# Autodesk Inventor assembly: 000.003 - Блок АКБ СБ
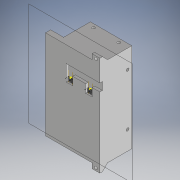
[picture p0: Inventor's stored thumbnail of the model, 180x180]
Saved by Autodesk Inventor 2022 (Build 260153000, 153)
## iProperties
Created: 2022-02-26
Part Number: 000.003 - Блок АКБ СБ
Document SubType Name: Assembly
Designer: Petrov Ivan
Author: Petrov Ivan
## Documents named in this file (4)
- C:\Users\Ivan Petrov\Documents\GitHub\OmniBot\design\000.003 - Блок АКБ СБ.iam
- C:\Users\Ivan Petrov\Documents\GitHub\OmniBot\design\000.003.001 - Основание.ipt
- C:\Users\Ivan Petrov\Documents\GitHub\OmniBot\design\standart_components\NUCLEO.ipt
- C:\Users\Ivan Petrov\Documents\GitHub\OmniBot\design\standart_components\connectrs\JST - XH - Thru (R) - 4Pin - 2.54mm.ipt
## Components (5 placed, 3 different names)
1. 000.003.001 - Основание.ipt:1 — Совмещение:2, Совмещение:3, Заподлицо:2, Совмещение:4, Совмещение:5, Заподлицо:3, Совмещение:6, Совмещение:7, Касательность:1, Касательность:2
2. NUCLEO.ipt:1 — Совмещение:6, Касательность:2, Заподлицо:4
3. NUCLEO.ipt:2 — Совмещение:7, Касательность:1, Заподлицо:4
4. JST - XH - Thru (R) - 4Pin - 2.54mm:1 — Совмещение:4, Совмещение:5, Заподлицо:3
5. JST - XH - Thru (R) - 4Pin - 2.54mm:2 — Совмещение:2, Совмещение:3, Заподлицо:2
## Relationships (11: Mate 6, Flush 3, Tangent 2)
- Совмещение:2 [Mate]: 000.003.001 - Основание.ipt:1 ↔ JST - XH - Thru (R) - 4Pin - 2.54mm:2
- Совмещение:3 [Mate]: 000.003.001 - Основание.ipt:1 ↔ JST - XH - Thru (R) - 4Pin - 2.54mm:2
- Заподлицо:2 [Flush]: 000.003.001 - Основание.ipt:1 ↔ JST - XH - Thru (R) - 4Pin - 2.54mm:2
- Совмещение:4 [Mate]: 000.003.001 - Основание.ipt:1 ↔ JST - XH - Thru (R) - 4Pin - 2.54mm:1
- Совмещение:5 [Mate]: 000.003.001 - Основание.ipt:1 ↔ JST - XH - Thru (R) - 4Pin - 2.54mm:1
- Заподлицо:3 [Flush]: 000.003.001 - Основание.ipt:1 ↔ JST - XH - Thru (R) - 4Pin - 2.54mm:1
- Совмещение:6 [Mate] (5 mm): 000.003.001 - Основание.ipt:1 ↔ NUCLEO.ipt:1
- Совмещение:7 [Mate] (5 mm): 000.003.001 - Основание.ipt:1 ↔ NUCLEO.ipt:2
- Касательность:1 [Tangent]: 000.003.001 - Основание.ipt:1 ↔ NUCLEO.ipt:2
- Касательность:2 [Tangent]: 000.003.001 - Основание.ipt:1 ↔ NUCLEO.ipt:1
- Заподлицо:4 [Flush]: NUCLEO.ipt:1 ↔ NUCLEO.ipt:2
